# Autodesk Inventor assembly: leg_ass_1_MIR
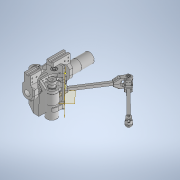
[picture p0: Inventor's stored thumbnail of the model, 180x180]
Saved by Autodesk Inventor 2020 (Build 240168000, 168)
## iProperties
Created: 2019-05-04
Part Number: leg_ass_1_MIR
Document SubType Name: Assembly
Designer: psrob
Author: psrob
## Documents named in this file (9)
- E:\projects-2\project dog gen2\hardware\leg_ass_1_MIR.iam
- E:\projects-2\project dog gen2\hardware\leg_bone_2_MIR.iam
- E:\projects-2\project dog gen2\hardware\leg_bone_1_MIR.iam
- E:\projects-2\project dog gen2\hardware\2GT_wheel_MIR.ipt
- E:\projects-2\project dog gen2\hardware\bearing_6_10_3_MIR.ipt
- E:\projects-2\project dog gen2\hardware\leg_motor_moudle_MIR.iam
- E:\projects-2\project dog gen2\hardware\dog_bone_1_MIR.ipt
- E:\projects-2\project dog gen2\hardware\motor_2_MIR.ipt
- E:\projects-2\project dog gen2\hardware\dog_bone_3_MIR1.ipt
## Components (9 placed, 8 different names)
1. leg_bone_2_MIR:1 [sub-assembly] — Insert:1, Insert:5, Insert:3, Insert:4, Insert:6
2. leg_bone_1_MIR:1 [sub-assembly] — Insert:1
3. 2GT_wheel_MIR:1 — Insert:5
4. bearing_6_10_3_MIR:1 — Insert:3
5. bearing_6_10_3_MIR:2 — Insert:4
6. leg_motor_moudle_MIR:1 [sub-assembly] — Insert:6, Insert:9, Insert:8
7. dog_bone_1_MIR:1 — Insert:9, Angle:1, Flush:1
8. motor_2_MIR:1 — Insert:8, Insert:10, Mate:1
9. dog_bone_3_MIR1:1 — Insert:10, Angle:1, Mate:1, Flush:1
## Relationships (11: Insert 8, Angle 1, Mate 1, Flush 1)
- Insert:1: leg_bone_2_MIR:1 ↔ leg_bone_1_MIR:1
- Insert:5 (0.5 mm): leg_bone_2_MIR:1 ↔ 2GT_wheel_MIR:1
- Insert:3: leg_bone_2_MIR:1 ↔ bearing_6_10_3_MIR:1
- Insert:4: leg_bone_2_MIR:1 ↔ bearing_6_10_3_MIR:2
- Insert:6 (0.5 mm): leg_bone_2_MIR:1 ↔ leg_motor_moudle_MIR:1
- Insert:9: leg_motor_moudle_MIR:1 ↔ dog_bone_1_MIR:1
- Insert:8 (-12 mm): leg_motor_moudle_MIR:1 ↔ motor_2_MIR:1
- Insert:10: motor_2_MIR:1 ↔ dog_bone_3_MIR1:1
- Angle:1 (0 deg): dog_bone_1_MIR:1 ↔ dog_bone_3_MIR1:1
- Mate:1: motor_2_MIR:1 ↔ dog_bone_3_MIR1:1
- Flush:1: dog_bone_1_MIR:1 ↔ dog_bone_3_MIR1:1
